# Autodesk Inventor assembly: LEG2
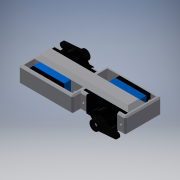
[picture p0: Inventor's stored thumbnail of the model, 180x180]
Saved by Autodesk Inventor 2017 (Build 210142000, 142)
## iProperties
Created: 2017-09-24
Part Number: LEG2
Document SubType Name: Assembly
Designer: Alexander Miller
Author: Alexander Miller
## Documents named in this file (4)
- D:\Daten\Documents\Git\HeRo-Mini\Hardware\LEG2.iam
- D:\Daten\Documents\Git\HeRo-Mini\Hardware\FEMUR2_A.ipt
- D:\Daten\Documents\Git\HeRo-Mini\Hardware\SERVO.iam
- D:\Daten\Documents\Git\HeRo-Mini\Hardware\FEMUR2_B.ipt
## Components (5 placed, 3 different names)
1. FEMUR2_A:1 — Rigid:1, Rigid:2
2. SERVO:1 [sub-assembly] — Rigid:1, Rigid:3
3. SERVO:2 [sub-assembly] — Rigid:2, Rigid:4
4. FEMUR2_B:1 — Rigid:3
5. FEMUR2_B:2 — Rigid:4
## Relationships (4: WeldJoint 4)
- Rigid:1 [WeldJoint]: FEMUR2_A:1 ↔ SERVO:1
- Rigid:2 [WeldJoint]: FEMUR2_A:1 ↔ SERVO:2
- Rigid:3 [WeldJoint]: SERVO:1 ↔ FEMUR2_B:1
- Rigid:4 [WeldJoint]: SERVO:2 ↔ FEMUR2_B:2
